# Autodesk Inventor assembly: wafel_rev4
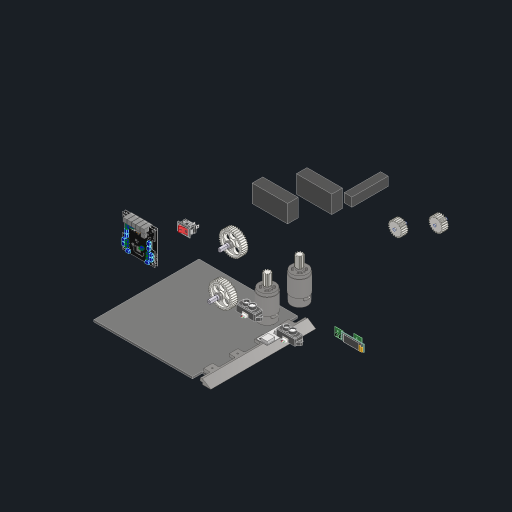
[picture p0: Inventor's stored thumbnail of the model, 512x512]
Saved by Autodesk Inventor 2023 (Build 270158000, 158)
## iProperties
Created: 2024-05-25
Part Number: wafel_rev4
Document SubType Name: Assembly
Designer: szymo
Mass: 531.086 g
Surface Area: 832.687 cm^2
Volume: 163.75 cm^3
Density: 3.24327 g/cm^3
Author: szymo
## iProperties of the stored document TFMINI_S_UART.ipt
Created: 2023-12-04
Part Number: TFMINI S UART
Material: Generic
Description: STEP AP214
Document SubType Name: Modeling
Designer: mateu
Density: 1 g/cm^3
Appearance: Default
Mass: 6.04913 g
Surface Area: 27.6076 cm^2
Volume: 6.04913 cm^3
Sending System: SolidWorks 2016
Preprocessor: SwSTEP 2.0
Title: TFMINI S UART.STEP
Author: USER
Revision Number: ANY
## Documents named in this file (17)
- D:\roboilo\robots\codename wafel - australia\3d_parts\rev4\wafel_rev4.iam
- **D:\roboilo\robots\codename wafel - australia\3d_parts\rev4\wafel_rev4.iam*LocalDocs*xAaaaqfaaAaaaaaaaAaaaqmipQa*TFMINI_S_UART.ipt
- D:\roboilo\robots\codename wafel - australia\3d_parts\rev4\128x32-OLED.ipt
- D:\roboilo\robots\codename wafel - australia\3d_parts\rev4\interface_board.ipt
- D:\roboilo\robots\codename wafel - australia\3d_parts\rev4\KTIR-Board.ipt
- D:\roboilo\robots\codename wafel - australia\3d_parts\rev4\motor_w_gear.iam
- D:\roboilo\robots\codename wafel - australia\3d_parts\rev4\plog.ipt
- D:\roboilo\robots\codename wafel - australia\3d_parts\rev4\rs390_w_gear.ipt
- D:\roboilo\robots\codename wafel - australia\3d_parts\rev4\smolgear_shaft.ipt
- D:\roboilo\robots\codename wafel - australia\3d_parts\rev4\stack.iam
- D:\roboilo\robots\codename wafel - australia\3d_parts\rev4\Switch.ipt
- D:\roboilo\robots\codename wafel - australia\3d_parts\rev4\wheel_axle.iam
- D:\roboilo\robots\codename wafel - australia\3d_parts\rev4\Design Accelerator\smolGear.iam
- D:\roboilo\robots\codename wafel - australia\3d_parts\rev4\lipo3s650mah.ipt
- D:\roboilo\robots\codename wafel - australia\3d_parts\rev4\lipo2s450mah.ipt
- D:\roboilo\robots\codename wafel - australia\3d_parts\rev4\base.ipt
- D:\roboilo\robots\codename wafel - australia\3d_parts\rev4\TFMINI_S_UART.ipt
## Components (22 placed, 15 different names)
1. base:1 — Mate:3, Mate:4, Flush:5
2. plog:1 — Mate:3, Mate:4, Flush:5
3. motor_w_gear:1 [sub-assembly]
4. wheel_axle:1 [sub-assembly]
5. smolGear:1 [sub-assembly] — Mate:1, Flush:3
6. smolgear_shaft:1 — Mate:1, Flush:3
7. motor_w_gear:2 [sub-assembly]
8. wheel_axle:2 [sub-assembly]
9. smolGear:2 [sub-assembly] — Mate:2, Flush:4
10. smolgear_shaft:2 — Mate:2, Flush:4
11. lipo3s650mah:1
12. lipo2s450mah:1
13. lipo3s650mah:2
14. KTIR-Board:1
15. KTIR-Board:2
16. TFMINI_S_UART:2
17. TFMINI_S_UART:1
18. 128x32-OLED:1
19. interface_board:1
20. rs390_w_gear:1
21. stack:1 [sub-assembly]
22. Switch:1
## Relationships (7: Mate 4, Flush 3)
- Mate:1: smolGear:1 ↔ smolgear_shaft:1
- Flush:3 (-2 mm): smolGear:1 ↔ smolgear_shaft:1
- Mate:2: smolGear:2 ↔ smolgear_shaft:2
- Flush:4 (-2 mm): smolGear:2 ↔ smolgear_shaft:2
- Mate:3: base:1 ↔ plog:1
- Mate:4: base:1 ↔ plog:1
- Flush:5: base:1 ↔ plog:1
